# Autodesk Inventor assembly: 01 MAIN ASM Ender_3
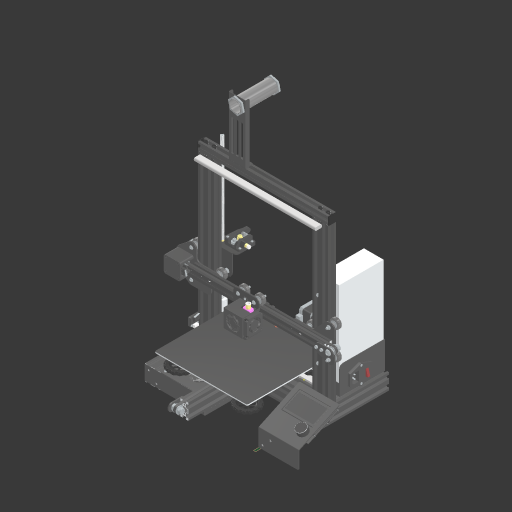
[picture p0: Inventor's stored thumbnail of the model, 512x512]
Saved by Autodesk Inventor 2023 (Build 270158000, 158)
## iProperties
Created: 2018-08-14
Part Number: 01 MAIN ASM Ender_3
Document SubType Name: Assembly
Designer: alber
Sending System: SolidWorks 2015
Last Author: Poseidon
Last Saved: 2018-08-17
Author: alber
## Documents named in this file (14)
- C:\Users\alber\Desktop\Ender-3 Parts\01 MAIN ASM Ender_3.iam
- C:\Users\alber\Desktop\Ender-3 Parts\ASM Frame.iam
- C:\Users\alber\Desktop\Ender-3 Parts\ASM X-Axis.iam
- C:\Users\alber\Desktop\Ender-3 Parts\ASM Y-Axis.iam
- C:\Users\alber\Desktop\Ender-3 Parts\ASM Z-Axis.iam
- C:\Users\alber\Desktop\Ender-3 Parts\ASM Display.iam
- C:\Users\alber\Desktop\Ender-3 Parts\ASM Electronic Enclosure.iam
- C:\Users\alber\Desktop\Ender-3 Parts\ASM Spool Holder.iam
- C:\Users\alber\Desktop\Ender-3 Parts\ASM Power Supply.iam
- C:\Users\alber\Desktop\Ender-3 Parts\Picase.ipt
- C:\Users\alber\Desktop\Ender-3 Parts\RaspberryPi 3 A+.iam
- C:\Users\alber\Desktop\Ender-3 Parts\LM2596 DC to DC Buck Converter 3 A\converterLM2596.iam
- C:\Users\alber\Desktop\Ender-3 Parts\Picover.ipt
- C:\Users\alber\Desktop\Led Light.ipt
## Components (14 placed, 13 different names)
1. ASM Frame:1 [sub-assembly] — Flush:1, Flush:2, Mate:7, Angle:1
2. ASM X-Axis:1 [sub-assembly]
3. ASM Y-Axis:1 [sub-assembly]
4. ASM Z-Axis:1 [sub-assembly]
5. ASM Display:1 [sub-assembly]
6. ASM Electronic Enclosure:1 [sub-assembly]
7. ASM Spool Holder:1 [sub-assembly]
8. ASM Power Supply:1 [sub-assembly]
9. Picase:1 — Flush:1, Flush:2, Mate:1, Mate:4, Mate:5, Mate:6, Flush:4, Flush:5
10. RaspberryPi 3 A+:1 [sub-assembly] — Mate:1
11. converterLM2596:1 [sub-assembly] — Mate:4, Flush:3
12. converterLM2596:2 [sub-assembly] — Mate:5, Mate:6, Flush:3
13. Picover:1 — Flush:4, Flush:5
14. Led Light:1 — Mate:7, Angle:1
## Relationships (11: Flush 5, Mate 5, Angle 1)
- Flush:1: ASM Frame:1 ↔ Picase:1
- Flush:2: ASM Frame:1 ↔ Picase:1
- Mate:1 (8 mm): Picase:1 ↔ RaspberryPi 3 A+:1
- Mate:4 (5 mm): Picase:1 ↔ converterLM2596:1
- Mate:5 (5 mm): Picase:1 ↔ converterLM2596:2
- Mate:6 (8 mm): Picase:1 ↔ converterLM2596:2
- Flush:3: converterLM2596:1 ↔ converterLM2596:2
- Flush:4: Picase:1 ↔ Picover:1
- Flush:5: Picase:1 ↔ Picover:1
- Mate:7: ASM Frame:1 ↔ Led Light:1
- Angle:1 (180 deg): ASM Frame:1 ↔ Led Light:1
